# Autodesk Inventor assembly: Hanging Dish Rack
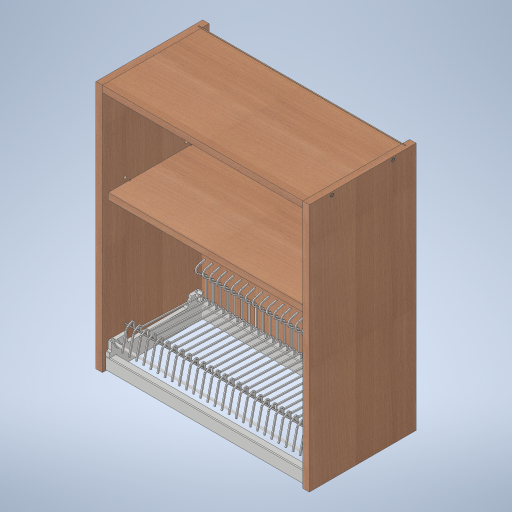
[picture p0: Inventor's stored thumbnail of the model, 512x512]
Saved by Autodesk Inventor 2024 (Build 280153000, 153)
## iProperties
RuleStatus: InUse
Created: 2017-01-23
Part Number: Hanging Dish Rack
Document SubType Name: Assembly
Designer: SvetlanaB
Author: SvetlanaB
## Documents named in this file (12)
- C:\W4INV 2024 Design\iBOX LIBRARY\Kitchen\Wall Cabinets\Dish Rack\Dish Rack.iam
- C:\W4INV 2024 Design\iBOX LIBRARY\Kitchen\Wall Cabinets\Dish Rack\Back panel.ipt
- C:\W4INV 2024 Design\iBOX LIBRARY\Kitchen\Wall Cabinets\Dish Rack\Right panel.ipt
- C:\W4INV 2024 Design\iBOX LIBRARY\Kitchen\Wall Cabinets\Dish Rack\Left panel.ipt
- C:\W4INV 2024 Design\iBOX LIBRARY\Kitchen\Wall Cabinets\Dish Rack\Top panel.ipt
- C:\W4INV 2024 Design\iBOX LIBRARY\Kitchen\Wall Cabinets\Dish Rack\Dish Rack Wire.iam
- C:\W4INV 2024 Design\_LIBRARY\Fixed joints\Confirmat\CONFIRMAT\Confirmat L50 NB T18 PB T 18.ipt
- C:\W4INV 2024 Design\iBOX LIBRARY\Kitchen\Wall Cabinets\Dish Rack\Dish Rack concept.ipt
- C:\W4INV 2024 Design\iBOX LIBRARY\Kitchen\Wall Cabinets\Dish Rack\Shelf.ipt
- C:\W4INV 2024 Design\_LIBRARY\Holders\Shelf holder D5\Shelf support D5 L16 with hole covers.ipt
- C:\W4INV 2023 Design\LIBRARY\Fixed joints\Confirmat\CONFIRMAT.ipt
- C:\W4INV 2023 Design\LIBRARY\Holders\Shelf holder D5.ipt
## Components (15 placed, 9 different names)
1. @Skeleton
2. Back panel:1
3. Right panel:1 — Flush:1, Flush:2, Nestled Board Plane:1, Nestled Board Plane:3, Side Board Plane:2, Side Board Plane:4
4. Left panel:1 — Nestled Board Plane:2, Nestled Board Plane:4, Side Board Plane:1, Side Board Plane:3
5. Top panel:1 — Pillar Board Side Plane:1, Pillar Board Side Plane:2, Pillar Board Side Plane:3, Pillar Board Side Plane:4
6. Dish Rack Wire:1 [sub-assembly]
7. Confirmat L50 NB T18 PB T 18:1 — Axis Plane:1, Nestled Board Plane:1, Pillar Board Side Plane:1
8. Confirmat L50 NB T18 PB T 18:2 — Axis Plane:2, Nestled Board Plane:2, Pillar Board Side Plane:2
9. Confirmat L50 NB T18 PB T 18:3 — Axis Plane:3, Nestled Board Plane:3, Pillar Board Side Plane:3
10. Confirmat L50 NB T18 PB T 18:4 — Axis Plane:4, Nestled Board Plane:4, Pillar Board Side Plane:4
11. Shelf:1 — Shelf Pottom Plane:1, Shelf Pottom Plane:2, Shelf Pottom Plane:3, Shelf Pottom Plane:4
12. Shelf support D5 L16 with hole covers:1 — Axis Plane:5, Side Board Plane:1, Shelf Pottom Plane:1
13. Shelf support D5 L16 with hole covers:2 — Axis Plane:6, Side Board Plane:2, Shelf Pottom Plane:2
14. Shelf support D5 L16 with hole covers:3 — Axis Plane:7, Side Board Plane:3, Shelf Pottom Plane:3
15. Shelf support D5 L16 with hole covers:4 — Axis Plane:8, Side Board Plane:4, Shelf Pottom Plane:4
## Relationships (26: Mate 20, Flush 6)
- Flush:1 (-64 mm): Right panel:1
- Flush:2 (-64 mm): Right panel:1
- Axis Plane:1 [Mate]: Confirmat L50 NB T18 PB T 18:1
- Nestled Board Plane:1 [Flush]: Right panel:1 ↔ Confirmat L50 NB T18 PB T 18:1
- Pillar Board Side Plane:1 [Mate] (-9 mm): Top panel:1 ↔ Confirmat L50 NB T18 PB T 18:1
- Axis Plane:2 [Mate]: Confirmat L50 NB T18 PB T 18:2
- Nestled Board Plane:2 [Flush]: Left panel:1 ↔ Confirmat L50 NB T18 PB T 18:2
- Pillar Board Side Plane:2 [Mate] (-9 mm): Top panel:1 ↔ Confirmat L50 NB T18 PB T 18:2
- Axis Plane:3 [Mate]: Confirmat L50 NB T18 PB T 18:3
- Nestled Board Plane:3 [Flush]: Right panel:1 ↔ Confirmat L50 NB T18 PB T 18:3
- Pillar Board Side Plane:3 [Mate] (-9 mm): Top panel:1 ↔ Confirmat L50 NB T18 PB T 18:3
- Axis Plane:4 [Mate]: Confirmat L50 NB T18 PB T 18:4
- Nestled Board Plane:4 [Flush]: Left panel:1 ↔ Confirmat L50 NB T18 PB T 18:4
- Pillar Board Side Plane:4 [Mate] (-9 mm): Top panel:1 ↔ Confirmat L50 NB T18 PB T 18:4
- Axis Plane:5 [Mate]: Shelf support D5 L16 with hole covers:1
- Side Board Plane:1 [Mate]: Left panel:1 ↔ Shelf support D5 L16 with hole covers:1
- Shelf Pottom Plane:1 [Mate] (2.5 mm): Shelf:1 ↔ Shelf support D5 L16 with hole covers:1
- Axis Plane:6 [Mate]: Shelf support D5 L16 with hole covers:2
- Side Board Plane:2 [Mate]: Right panel:1 ↔ Shelf support D5 L16 with hole covers:2
- Shelf Pottom Plane:2 [Mate] (2.5 mm): Shelf:1 ↔ Shelf support D5 L16 with hole covers:2
- Axis Plane:7 [Mate]: Shelf support D5 L16 with hole covers:3
- Side Board Plane:3 [Mate]: Left panel:1 ↔ Shelf support D5 L16 with hole covers:3
- Shelf Pottom Plane:3 [Mate] (2.5 mm): Shelf:1 ↔ Shelf support D5 L16 with hole covers:3
- Axis Plane:8 [Mate]: Shelf support D5 L16 with hole covers:4
- Side Board Plane:4 [Mate]: Right panel:1 ↔ Shelf support D5 L16 with hole covers:4
- Shelf Pottom Plane:4 [Mate] (2.5 mm): Shelf:1 ↔ Shelf support D5 L16 with hole covers:4
## Named parameters: Panel_thickness = 18 mm, Height = 360 mm, Width = 600 mm, Depth = 300 mm, Shelf_Space_From_Top = 250 mm
